# Autodesk Inventor assembly: Arm Assembly
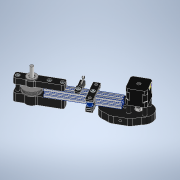
[picture p0: Inventor's stored thumbnail of the model, 180x180]
Saved by Autodesk Inventor 2022 (Build 260153000, 153)
## iProperties
Created: 2022-04-09
Part Number: Arm Assembly
Document SubType Name: Assembly
Designer: JK
Author: JK
## Documents named in this file (24)
- C:\Users\JK\Documents\Inventor\ScaraNema\SCARA-3DP\Parts\Arm\Arm Assembly.iam
- C:\Users\JK\Documents\Inventor\ScaraNema\SCARA-3DP\Parts\Arm\Arm platform.ipt
- C:\Users\JK\Documents\Inventor\ScaraNema\SCARA-3DP\Parts\Common components\Motor.ipt
- C:\Users\JK\Documents\Inventor\ScaraNema\SCARA-3DP\Parts\Arm\Arm motor spacer.ipt
- C:\Users\JK\Documents\Inventor\ScaraNema\SCARA-3DP\Parts\Fasteners\M3x35 socket bolt.ipt
- C:\Users\JK\Documents\Inventor\ScaraNema\SCARA-3DP\Parts\Common components\GT2 16 Pulley.ipt
- C:\Users\JK\Documents\Inventor\ScaraNema\SCARA-3DP\Parts\Common components\V-Slot 20x20\V-Slot 20x20x150.ipt
- C:\Users\JK\Documents\Inventor\ScaraNema\SCARA-3DP\Parts\V-Slot 20x20.ipt
- C:\Users\JK\Documents\Inventor\ScaraNema\SCARA-3DP\Parts\Arm\Belt tensor.ipt
- C:\Users\JK\Documents\Inventor\ScaraNema\SCARA-3DP\Parts\Common components\Idle pulley 16\GT2-16 Idle pulley.iam
- C:\Users\JK\Documents\Inventor\ScaraNema\SCARA-3DP\Parts\Fasteners\M3x25 socket solt.ipt
- C:\Users\JK\Documents\Inventor\ScaraNema\SCARA-3DP\Parts\Fasteners\M3 Hex nut.ipt
- C:\Users\JK\Documents\Inventor\ScaraNema\SCARA-3DP\Parts\Fasteners\M5x8 Flat head bolt.ipt
- C:\Users\JK\Documents\Inventor\ScaraNema\SCARA-3DP\Parts\Fasteners\M5x20 Flat head bolt.ipt
- C:\Users\JK\Documents\Inventor\ScaraNema\SCARA-3DP\Parts\Fasteners\M5 Hex nut.ipt
- C:\Users\JK\Documents\Inventor\ScaraNema\SCARA-3DP\Parts\Fasteners\M5x10 set screw.ipt
- C:\Users\JK\Documents\Inventor\ScaraNema\SCARA-3DP\Parts\Fasteners\M5 T-Nut Drop-in 20x20.ipt
- C:\Users\JK\Documents\Inventor\ScaraNema\SCARA-3DP\Parts\Arm\Elbow assembly.iam
- C:\Users\JK\Documents\Inventor\ScaraNema\SCARA-3DP\Parts\Common components\Limit switch.ipt
- C:\Users\JK\Documents\Inventor\ScaraNema\SCARA-3DP\Parts\Fasteners\M2x10 socket bolt.ipt
- C:\Users\JK\Documents\Inventor\ScaraNema\SCARA-3DP\Parts\Fasteners\M2 Hex nut.ipt
- C:\Users\JK\Documents\Inventor\ScaraNema\SCARA-3DP\Parts\Arm\Pulley support separator.ipt
- C:\Users\JK\Documents\Inventor\ScaraNema\SCARA-3DP\Parts\Arm\yendstop.ipt
- C:\Users\JK\Documents\Inventor\ScaraNema\SCARA-3DP\Parts\Fasteners\M5x10 Flat head bolt.ipt
## Components (39 placed, 22 different names)
1. Arm platform:1
2. Motor:1
3. GT2 16 Pulley:1
4. V-Slot 20x20x150:1 — Coincidencia:36, Nivelación:12, Coincidencia:37, Coincidencia:55, Nivelación:17, Ángulo:9
5. Belt tensor:1
6. GT2-16 Idle pulley:1 [sub-assembly]
7. GT2-16 Idle pulley:2 [sub-assembly]
8. M3x25 socket solt:1
9. M3x25 socket solt:2
10. M3 Hex nut:1
11. M3 Hex nut:2
12. M5x8 Flat head bolt:1
13. M5x20 Flat head bolt:1
14. M5x20 Flat head bolt:2
15. M5 Hex nut:1
16. M5 Hex nut:2
17. M5x10 set screw:1
18. M5x10 set screw:2
19. M5 T-Nut Drop-in 20x20:1
20. M5 T-Nut Drop-in 20x20:2
21. M5 T-Nut Drop-in 20x20:3
22. Elbow assembly:1 [sub-assembly] — Coincidencia:36, Nivelación:12, Coincidencia:37, Coincidencia:53, Coincidencia:54
23. Limit switch:1 — Coincidencia:47, Coincidencia:48, Coincidencia:49, Ángulo:9, Coincidencia:57
24. M2x10 socket bolt:1 — Coincidencia:47, Nivelación:15, Coincidencia:49, Coincidencia:50
25. M2x10 socket bolt:2 — Coincidencia:48, Nivelación:15, Coincidencia:51, Coincidencia:56
26. M2 Hex nut:1 — Coincidencia:50, Ángulo:8, Nivelación:16, Coincidencia:58
27. M2 Hex nut:2 — Coincidencia:51, Ángulo:8, Nivelación:16, Ángulo:10
28. Pulley support separator:1 — Coincidencia:53, Coincidencia:54
29. yendstop:1 — Coincidencia:55, Nivelación:17, Coincidencia:56, Coincidencia:57, Coincidencia:58, Ángulo:10, Coincidencia:59, Coincidencia:60, Coincidencia:62
30. M5x10 Flat head bolt:1 — Coincidencia:59, Coincidencia:60, Coincidencia:61
31. M5 T-Nut Drop-in 20x20:4 — Coincidencia:61, Coincidencia:62
32. Arm motor spacer:1
33. M3x35 socket bolt:1
34. M3x35 socket bolt:2
35. Arm motor spacer:2
36. M3x35 socket bolt:3
37. Arm motor spacer:3
38. M3x35 socket bolt:4
39. Arm motor spacer:4
## Component patterns: (4 elements, first: Arm motor spacer:1 + M3x35 socket bolt:1)
## Relationships (74: Mate 49, Flush 15, Angle 10)
- [Mate]: Arm platform:1 ↔ Arm motor spacer:1
- [Mate]: Arm platform:1 ↔ Arm motor spacer:1
- [Mate]: Motor:1 ↔ Arm motor spacer:1
- [Mate]: Arm motor spacer:1 ↔ M3x35 socket bolt:1
- [Mate]: Arm platform:1 ↔ M3x35 socket bolt:1
- [Mate]: Motor:1 ↔ GT2 16 Pulley:1
- [Flush] (-6.25 mm): Arm platform:1 ↔ GT2 16 Pulley:1
- [Angle] (90 deg): Arm platform:1 ↔ Motor:1
- [Mate]: Arm platform:1 ↔ Motor:1
- [Mate]: Arm platform:1 ↔ V-Slot 20x20x150:1
- [Flush] (-25 mm): Arm platform:1 ↔ V-Slot 20x20x150:1
- [Mate] (10 mm): Motor:1 ↔ V-Slot 20x20x150:1
- [Mate] (0.15 mm): V-Slot 20x20x150:1 ↔ Belt tensor:1
- [Mate] (0.15 mm): V-Slot 20x20x150:1 ↔ Belt tensor:1
- [Flush] (-50 mm): V-Slot 20x20x150:1 ↔ Belt tensor:1
- [Mate]: Belt tensor:1 ↔ GT2-16 Idle pulley:1
- [Mate]: Belt tensor:1 ↔ GT2-16 Idle pulley:2
- [Flush]: GT2-16 Idle pulley:1 ↔ GT2-16 Idle pulley:2
- [Mate] (4 mm): Belt tensor:1 ↔ GT2-16 Idle pulley:1
- [Flush]: M3x25 socket solt:1 ↔ M3x25 socket solt:2
- [Mate]: M3x25 socket solt:1 ↔ M3 Hex nut:2
- [Angle] (0 deg): Belt tensor:1 ↔ M3 Hex nut:2
- [Mate]: M3x25 socket solt:2 ↔ M3 Hex nut:1
- [Angle] (0 deg): Belt tensor:1 ↔ M3 Hex nut:1
- [Mate]: Belt tensor:1 ↔ M3 Hex nut:1
- [Flush]: M3 Hex nut:1 ↔ M3 Hex nut:2
- [Mate]: Belt tensor:1 ↔ M5x8 Flat head bolt:1
- [Mate]: Belt tensor:1 ↔ M5x8 Flat head bolt:1
- [Mate]: Arm platform:1 ↔ M5x20 Flat head bolt:1
- [Mate]: Arm platform:1 ↔ M5x20 Flat head bolt:1
- [Mate]: Arm platform:1 ↔ M5x20 Flat head bolt:2
- [Flush]: M5x20 Flat head bolt:1 ↔ M5x20 Flat head bolt:2
- [Mate]: Arm platform:1 ↔ M5 Hex nut:1
- [Mate]: Arm platform:1 ↔ M5 Hex nut:2
- [Angle] (0 deg): Motor:1 ↔ M5 Hex nut:2
- [Flush]: M5 Hex nut:1 ↔ M5 Hex nut:2
- [Mate]: Arm platform:1 ↔ M5 Hex nut:1
- [Mate]: Arm platform:1 ↔ M5 Hex nut:2
- [Mate]: Arm platform:1 ↔ M5x10 set screw:1
- [Mate]: Arm platform:1 ↔ M5x10 set screw:2
- [Mate]: M5x20 Flat head bolt:2 ↔ M5 T-Nut Drop-in 20x20:1
- [Mate]: M5x20 Flat head bolt:1 ↔ M5 T-Nut Drop-in 20x20:2
- [Flush]: M5 T-Nut Drop-in 20x20:1 ↔ M5 T-Nut Drop-in 20x20:2
- [Angle] (0 deg): Belt tensor:1 ↔ M5 T-Nut Drop-in 20x20:2
- [Angle] (0 deg): M5 T-Nut Drop-in 20x20:1 ↔ M5 T-Nut Drop-in 20x20:2
- [Flush]: M5x20 Flat head bolt:2 ↔ M5 T-Nut Drop-in 20x20:1
- [Flush]: M5 T-Nut Drop-in 20x20:1 ↔ M5 T-Nut Drop-in 20x20:2
- [Mate]: M5x8 Flat head bolt:1 ↔ M5 T-Nut Drop-in 20x20:3
- [Angle] (0 deg): Belt tensor:1 ↔ M5 T-Nut Drop-in 20x20:3
- [Mate] (0.6 mm): Belt tensor:1 ↔ M5 T-Nut Drop-in 20x20:3
- Coincidencia:36 [Mate]: V-Slot 20x20x150:1 ↔ Elbow assembly:1
- Nivelación:12 [Flush]: V-Slot 20x20x150:1 ↔ Elbow assembly:1
- Coincidencia:37 [Mate] (-40 mm): V-Slot 20x20x150:1 ↔ Elbow assembly:1
- Coincidencia:47 [Mate]: Limit switch:1 ↔ M2x10 socket bolt:1
- Coincidencia:48 [Mate]: Limit switch:1 ↔ M2x10 socket bolt:2
- Nivelación:15 [Flush]: M2x10 socket bolt:1 ↔ M2x10 socket bolt:2
- Coincidencia:49 [Mate]: Limit switch:1 ↔ M2x10 socket bolt:1
- Coincidencia:50 [Mate]: M2x10 socket bolt:1 ↔ M2 Hex nut:1
- Coincidencia:51 [Mate]: M2x10 socket bolt:2 ↔ M2 Hex nut:2
- Ángulo:8 [Angle] (0 deg): M2 Hex nut:1 ↔ M2 Hex nut:2
- Nivelación:16 [Flush]: M2 Hex nut:1 ↔ M2 Hex nut:2
- Coincidencia:53 [Mate]: Elbow assembly:1 ↔ Pulley support separator:1
- Coincidencia:54 [Mate]: Elbow assembly:1 ↔ Pulley support separator:1
- Coincidencia:55 [Mate]: V-Slot 20x20x150:1 ↔ yendstop:1
- Nivelación:17 [Flush]: V-Slot 20x20x150:1 ↔ yendstop:1
- Coincidencia:56 [Mate]: M2x10 socket bolt:2 ↔ yendstop:1
- Ángulo:9 [Angle] (0 deg): V-Slot 20x20x150:1 ↔ Limit switch:1
- Coincidencia:57 [Mate]: Limit switch:1 ↔ yendstop:1
- Coincidencia:58 [Mate]: M2 Hex nut:1 ↔ yendstop:1
- Ángulo:10 [Angle] (0 deg): M2 Hex nut:2 ↔ yendstop:1
- Coincidencia:59 [Mate]: yendstop:1 ↔ M5x10 Flat head bolt:1
- Coincidencia:60 [Mate]: yendstop:1 ↔ M5x10 Flat head bolt:1
- Coincidencia:61 [Mate]: M5x10 Flat head bolt:1 ↔ M5 T-Nut Drop-in 20x20:4
- Coincidencia:62 [Mate] (1 mm): yendstop:1 ↔ M5 T-Nut Drop-in 20x20:4
## Named parameters: d11_d41 = 0 mm, d12_d42 = 0 mm, d13_d45 = 0 mm, d14_d46 = 0 mm, d15_d47 = 0 mm, d16_d48 = 90 deg, d17_d49 = 4, d19_d50 = 0 mm, d20_d51 = -6.25 mm, d21_d52 = 90 deg, d22_d53 = 0 mm, d23_d54 = 0 mm, d24_d55 = -25 mm
